# Autodesk Inventor assembly: CONTROLLER FINAL
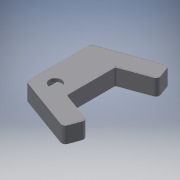
[picture p0: Inventor's stored thumbnail of the model, 180x180]
Saved by Autodesk Inventor 2019.4 (Build 234330000, 330)
## iProperties
Created: 2019-06-21
Part Number: CONTROLLER FINAL
Document SubType Name: Assembly
Designer: abdel
Author: abdel
## Documents named in this file (3)
- C:\Users\abdel\Downloads\10% project (laptop)-20190621T144919Z-001\10_ project (laptop)\drone\drone inventor\CONTROLLER FINAL.iam
- C:\Users\abdel\Downloads\10% project (laptop)-20190621T144919Z-001\10_ project (laptop)\drone\drone inventor\CONTROLLER CASE.ipt
- C:\Users\abdel\Downloads\10% project (laptop)-20190621T144919Z-001\10_ project (laptop)\drone\drone inventor\controller.ipt
## Components (2 placed, 2 different names)
1. CONTROLLER CASE:1 — Flush:1, Mate:1, Mate:2
2. controller:1 — Flush:1, Mate:1, Mate:2
## Relationships (3: Mate 2, Flush 1)
- Flush:1: CONTROLLER CASE:1 ↔ controller:1
- Mate:1: CONTROLLER CASE:1 ↔ controller:1
- Mate:2: CONTROLLER CASE:1 ↔ controller:1
